# Autodesk Inventor assembly: fuselage_motor_interface_assembly
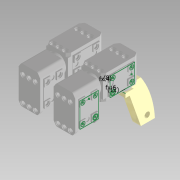
[picture p0: Inventor's stored thumbnail of the model, 180x180]
Saved by Autodesk Inventor 2021 (Build 250183000, 183)
## iProperties
Created: 2020-11-21
Part Number: fuselage_motor_interface_assembly
Document SubType Name: Assembly
Designer: Paco
Mass: 73.6057 g
Surface Area: 273.467 cm^2
Volume: 72.8792 cm^3
Density: 1.00997 g/cm^3
Author: Paco
## Documents named in this file (4)
- C:\Users\Kanenas\Desktop\IISRD_CAD_V\IISRD_V_v1\fuselage_motor_interface_assembly.iam
- C:\Users\Kanenas\Desktop\IISRD_CAD_V\IISRD_V_v1\motor assembly_v2_MIR.iam
- C:\Users\Kanenas\Desktop\IISRD_CAD_V\IISRD_V_v1\motor_elytra_interface.ipt
- C:\Users\Kanenas\Desktop\IISRD_CAD_V\IISRD_V_v1\motor assembly_v2_MIR_MIR1.iam
## Components (3 placed, 3 different names)
1. motor assembly_v2_MIR:1 [sub-assembly] — Mate:6, Rotational:1
2. motor_elytra_interface:1 — Mate:6, Rotational:1
3. motor assembly_v2_MIR_MIR1:1 [sub-assembly]
## Relationships (2: Mate 1, RevoluteJoint 1)
- Mate:6: motor assembly_v2_MIR:1 ↔ motor_elytra_interface:1
- Rotational:1 [RevoluteJoint]: motor assembly_v2_MIR:1 ↔ motor_elytra_interface:1
